# Autodesk Inventor assembly: WJ_0.09inGussetPuzzle
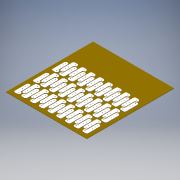
[picture p0: Inventor's stored thumbnail of the model, 180x180]
Saved by Autodesk Inventor 2018.3 (Build 223284000, 284)
## iProperties
Created: 2020-02-29
Part Number: WJ_0.09inGussetPuzzle
Document SubType Name: Assembly
Designer: 22barlalex
Author: 22barlalex
## Documents named in this file (4)
- C:\Users\22barlalex\Documents\GrabCAD\Infinite Recharge 2020\Build season\WJ_0.09inGussetPuzzle.iam
- C:\Users\22barlalex\Documents\GrabCAD\Infinite Recharge 2020\Build season\WJ_CLB_0.09inPlate.ipt
- C:\Users\22barlalex\Documents\GrabCAD\Infinite Recharge 2020\Build season\CLB_027_LifterBracket.ipt
- CLB_027_LifterBracket.ipt
## Components (52 placed, 2 different names)
1. WJ_CLB_0.09inPlate:1 — Mate:6, Mate:8, Flush:1, Flush:2, Mate:11, Mate:12
2. CLB_027_LifterBracket:1 — Mate:6, Mate:9, Mate:10, Flush:1, Flush:2
3. CLB_027_LifterBracket:2 — Mate:8, Mate:9, Mate:10
4. CLB_027_LifterBracket:3
5. CLB_027_LifterBracket:4
6. CLB_027_LifterBracket:5
7. CLB_027_LifterBracket:6
8. CLB_027_LifterBracket:7
9. CLB_027_LifterBracket:8
10. CLB_027_LifterBracket:9
11. CLB_027_LifterBracket:10
12. CLB_027_LifterBracket:11
13. CLB_027_LifterBracket:12
14. CLB_027_LifterBracket:13
15. CLB_027_LifterBracket:14
16. CLB_027_LifterBracket:15 — Flush:3
17. CLB_027_LifterBracket:16 — Mate:13
18. CLB_027_LifterBracket:17
19. CLB_027_LifterBracket:18
20. CLB_027_LifterBracket:19
21. CLB_027_LifterBracket:20
22. CLB_027_LifterBracket:21
23. CLB_027_LifterBracket:22
24. CLB_027_LifterBracket:23
25. CLB_027_LifterBracket:24
26. CLB_027_LifterBracket:25
27. CLB_027_LifterBracket:26
28. CLB_027_LifterBracket:27
29. CLB_027_LifterBracket:28
30. CLB_027_LifterBracket:29
31. CLB_027_LifterBracket:30
32. CLB_027_LifterBracket:31
33. CLB_027_LifterBracket:32
34. CLB_027_LifterBracket:33
35. CLB_027_LifterBracket:34
36. CLB_027_LifterBracket:35
37. CLB_027_LifterBracket:36
38. CLB_027_LifterBracket:37
39. CLB_027_LifterBracket:38
40. CLB_027_LifterBracket:39
41. CLB_027_LifterBracket:40
42. CLB_027_LifterBracket:41
43. CLB_027_LifterBracket:42
44. CLB_027_LifterBracket:43
45. CLB_027_LifterBracket:44
46. CLB_027_LifterBracket:45
47. CLB_027_LifterBracket:46
48. CLB_027_LifterBracket:47
49. CLB_027_LifterBracket:48
50. CLB_027_LifterBracket:49 — Mate:11, Mate:12, Mate:13, Flush:3
51. CLB_027_LifterBracket:50
52. CLB_027_LifterBracket:51
## Component patterns: (24 elements, first: CLB_027_LifterBracket:1 + CLB_027_LifterBracket:2), (3 elements, first: CLB_027_LifterBracket:49)
## Relationships (10: Mate 7, Flush 3)
- Mate:6: WJ_CLB_0.09inPlate:1 ↔ CLB_027_LifterBracket:1
- Mate:8: WJ_CLB_0.09inPlate:1 ↔ CLB_027_LifterBracket:2
- Mate:9 (5.08 mm): CLB_027_LifterBracket:1 ↔ CLB_027_LifterBracket:2
- Mate:10 (30.48 mm): CLB_027_LifterBracket:1 ↔ CLB_027_LifterBracket:2
- Flush:1 (25.4 mm): WJ_CLB_0.09inPlate:1 ↔ CLB_027_LifterBracket:1
- Flush:2 (25.4 mm): WJ_CLB_0.09inPlate:1 ↔ CLB_027_LifterBracket:1
- Mate:11: WJ_CLB_0.09inPlate:1 ↔ CLB_027_LifterBracket:49
- Mate:12: WJ_CLB_0.09inPlate:1 ↔ CLB_027_LifterBracket:49
- Mate:13 (5.08 mm): CLB_027_LifterBracket:16 ↔ CLB_027_LifterBracket:49
- Flush:3: CLB_027_LifterBracket:15 ↔ CLB_027_LifterBracket:49
